# Autodesk Inventor assembly: WheelWithPulley
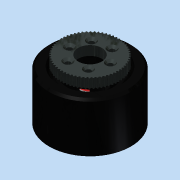
[picture p0: Inventor's stored thumbnail of the model, 180x180]
Saved by Autodesk Inventor 2015 (Build 190159000, 159)
## iProperties
Created: 2015-11-06
Part Number: WheelWithPulley
Document SubType Name: Assembly
Designer: Raphael
Author: Raphael
## Documents named in this file (3)
- \\psf\Home\Documents\electric-skateboard\CAD\WheelWithPulley.iam
- \\psf\Home\Documents\electric-skateboard\CAD\WheelWithBearing.iam
- \\psf\Home\Documents\electric-skateboard\CAD\WheelPulleyAssembly.iam
## Components (2 placed, 2 different names)
1. WheelWithBearing:1 [sub-assembly] — Mate:1, Mate:2
2. WheelPulleyAssembly:1 [sub-assembly] — Mate:1, Mate:2
## Relationships (2: Mate 2)
- Mate:1: WheelWithBearing:1 ↔ WheelPulleyAssembly:1
- Mate:2 (0.5 mm): WheelWithBearing:1 ↔ WheelPulleyAssembly:1
